# Autodesk Inventor assembly: z_pulley
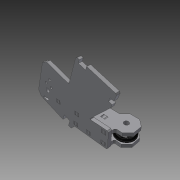
[picture p0: Inventor's stored thumbnail of the model, 180x180]
Saved by Autodesk Inventor 2014 (Build 180170000, 170)
## iProperties
Created: 2014-04-03
Part Number: z_pulley
Document SubType Name: Assembly
Designer: buben
Author: buben
## Documents named in this file (7)
- C:\Users\buben\Documents\GitHub\bacon\inventor files\assemblies\z_pulley.iam
- C:\Users\buben\Documents\GitHub\bacon\inventor files\printer parts\z_axis_top_pulleys.ipt
- C:\Users\buben\Documents\GitHub\bacon\inventor files\printer parts\z_pulley_holder_left.ipt
- C:\Users\buben\Documents\GitHub\bacon\inventor files\printer parts\z_axis_top_cap.ipt
- C:\Users\buben\Documents\GitHub\bacon\inventor files\utils\rope_pulley.ipt
- C:\Users\buben\Documents\GitHub\bacon\inventor files\printer parts\z_pulley_holder.ipt
- C:\Users\buben\Documents\GitHub\bacon\inventor files\printer parts\z_pulley_holder_right.ipt
## Components (7 placed, 6 different names)
1. z_axis_top_pulleys:1 — Mate:1, Flush:1, Flush:2, Mate:2, Mate:3, Mate:4, Mate:11, Mate:12, Mate:16
2. z_pulley_holder_left:1 — Mate:1, Flush:1, Flush:2, Mate:6, Mate:7, Mate:8, Mate:9, Mate:14, Mate:15
3. z_axis_top_cap:1 — Mate:2, Mate:3, Mate:4
4. rope_pulley:1 — Mate:6, Mate:8
5. rope_pulley:2 — Mate:7, Mate:9
6. z_pulley_holder:1 — Mate:11, Mate:13, Mate:14, Mate:15
7. z_pulley_holder_right:1 — Mate:12, Mate:13, Mate:16
## Relationships (16: Mate 14, Flush 2)
- Mate:1: z_axis_top_pulleys:1 ↔ z_pulley_holder_left:1
- Flush:1: z_axis_top_pulleys:1 ↔ z_pulley_holder_left:1
- Flush:2 (3 mm): z_axis_top_pulleys:1 ↔ z_pulley_holder_left:1
- Mate:2: z_axis_top_pulleys:1 ↔ z_axis_top_cap:1
- Mate:3: z_axis_top_pulleys:1 ↔ z_axis_top_cap:1
- Mate:4: z_axis_top_pulleys:1 ↔ z_axis_top_cap:1
- Mate:6: z_pulley_holder_left:1 ↔ rope_pulley:1
- Mate:7: z_pulley_holder_left:1 ↔ rope_pulley:2
- Mate:8: z_pulley_holder_left:1 ↔ rope_pulley:1
- Mate:9: z_pulley_holder_left:1 ↔ rope_pulley:2
- Mate:11 (10 mm): z_axis_top_pulleys:1 ↔ z_pulley_holder:1
- Mate:12: z_axis_top_pulleys:1 ↔ z_pulley_holder_right:1
- Mate:13: z_pulley_holder:1 ↔ z_pulley_holder_right:1
- Mate:14: z_pulley_holder_left:1 ↔ z_pulley_holder:1
- Mate:15: z_pulley_holder_left:1 ↔ z_pulley_holder:1
- Mate:16: z_axis_top_pulleys:1 ↔ z_pulley_holder_right:1
